# Autodesk Inventor assembly: RollerAssembly
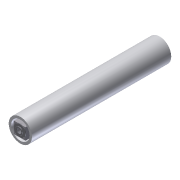
[picture p0: Inventor's stored thumbnail of the model, 180x180]
Saved by Autodesk Inventor 2012 (Build 160160000, 160)
## iProperties
Created: 2012-01-10
Part Number: RollerAssembly
Document SubType Name: Assembly
Designer: JesseK
Mass: 440.135 g
Surface Area: 1168.6 cm^2
Volume: 260.657 cm^3
Density: 1.68856 g/cm^3
Author: JesseK
## Documents named in this file (4)
- Z:\UserData\Documents\Inventor\team1885frc\Robot2012\Conveyor\RollerAssembly.iam
- Z:\UserData\Documents\Inventor\team1885frc\Robot2012\Conveyor\Conveyor_Roller_PVCPipe_size1.5.ipt
- Z:\UserData\Documents\Inventor\team1885frc\Robot2012\Conveyor\Conveyor_Roller_BearingMount.ipt
- Z:\UserData\Documents\Inventor\team1885frc\Hardware\Bearings\Bearing_0.375ID_0.875OD_flanged.ipt
## Components (5 placed, 3 different names)
1. Conveyor_Roller_PVCPipe_size1.5:1 — Mate:2, Mate:3, Mate:5, Mate:6
2. Conveyor_Roller_BearingMount:1 — Tangent:1, Tangent:2, Mate:1
3. Conveyor_Roller_BearingMount:2 — Tangent:3, Tangent:4, Mate:4
4. Bearing_0.375ID_0.875OD_flanged:1 — Tangent:1, Tangent:2, Mate:1, Mate:2, Mate:3
5. Bearing_0.375ID_0.875OD_flanged:2 — Tangent:3, Tangent:4, Mate:4, Mate:5, Mate:6
## Relationships (10: Mate 6, Tangent 4)
- Tangent:1: Conveyor_Roller_BearingMount:1 ↔ Bearing_0.375ID_0.875OD_flanged:1
- Tangent:2: Conveyor_Roller_BearingMount:1 ↔ Bearing_0.375ID_0.875OD_flanged:1
- Mate:1: Conveyor_Roller_BearingMount:1 ↔ Bearing_0.375ID_0.875OD_flanged:1
- Mate:2: Conveyor_Roller_PVCPipe_size1.5:1 ↔ Bearing_0.375ID_0.875OD_flanged:1
- Mate:3: Conveyor_Roller_PVCPipe_size1.5:1 ↔ Bearing_0.375ID_0.875OD_flanged:1
- Tangent:3: Conveyor_Roller_BearingMount:2 ↔ Bearing_0.375ID_0.875OD_flanged:2
- Tangent:4: Conveyor_Roller_BearingMount:2 ↔ Bearing_0.375ID_0.875OD_flanged:2
- Mate:4: Conveyor_Roller_BearingMount:2 ↔ Bearing_0.375ID_0.875OD_flanged:2
- Mate:5: Conveyor_Roller_PVCPipe_size1.5:1 ↔ Bearing_0.375ID_0.875OD_flanged:2
- Mate:6: Conveyor_Roller_PVCPipe_size1.5:1 ↔ Bearing_0.375ID_0.875OD_flanged:2
